# Autodesk Inventor assembly: Ark Test
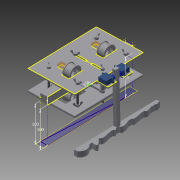
[picture p0: Inventor's stored thumbnail of the model, 180x180]
Saved by Autodesk Inventor 2015 (Build 190159000, 159)
## iProperties
Created: 2018-12-21
Part Number: Ark Test
Document SubType Name: Assembly
Designer: kostya
Author: kostya
## Documents named in this file (12)
- C:\Users\kostya\source\repos\Models\Arkanoid\Ark.ipt\Ark Test.iam
- C:\Users\kostya\source\repos\Models\Arkanoid\Ark.ipt\Top.ipt
- C:\Users\kostya\source\repos\Models\Arkanoid\Ark.ipt\Down.ipt
- C:\Users\kostya\source\repos\Models\Arkanoid\Ark.ipt\Screw.ipt
- C:\Users\kostya\source\repos\Models\Arkanoid\Ark.ipt\Stick.ipt
- C:\Users\kostya\source\repos\Models\Arkanoid\Ark.ipt\Nut.ipt
- C:\Users\kostya\source\repos\Models\Arkanoid\Ark.ipt\Screwk.ipt
- C:\Users\kostya\source\repos\Models\Arkanoid\Ather\ipt\Motors\Servo.ipt
- C:\Users\kostya\source\repos\Models\Arkanoid\Ather\ipt\Motors\Line for servo.ipt
- C:\Users\kostya\source\repos\Models\Arkanoid\Ark.ipt\Wheel.ipt
- C:\Users\kostya\source\repos\Models\Arkanoid\Ark.ipt\Kick.ipt
- C:\Users\kostya\source\repos\Models\Arkanoid\Ark.ipt\Nozzle.ipt
## Components (43 placed, 11 different names)
1. Kick:1 — Вставка:59, Вставка:60, Вставка:61, Вставка:62, Вставка:63, Вставка:64, Вставка:65
2. Nozzle:1 — Вставка:65
3. Top:1 — Вставка:1, Вставка:6, Вставка:7, Вставка:8, Вставка:9, Вставка:15, Вставка:16, Заподлицо:2, Вставка:21, Вставка:22, Вставка:23, Вставка:24, Вставка:46, Вставка:48, Вставка:50, Вставка:51, Вставка:52, Вставка:54, Вставка:55, Заподлицо:7, Совмещение:1, Совмещение:2, Заподлицо:8, Совмещение:3, Совмещение:4
4. Down:1 — Вставка:2, Вставка:3, Вставка:4, Вставка:5, Вставка:10, Вставка:11, Вставка:12, Вставка:13, Заподлицо:1, Заподлицо:2, Вставка:25, Вставка:26, Вставка:27, Вставка:28, Касательность:1, Заподлицо:3, Вставка:47, Вставка:49, Вставка:56, Вставка:57
5. Stick:1 — Заподлицо:1, Касательность:1, Заподлицо:3, Касательность:2, Заподлицо:5, Касательность:3, Касательность:4, Заподлицо:6
6. Nut:1 — Вставка:1, Вставка:36
7. Nut:2 — Вставка:7, Вставка:51
8. Nut:3 — Вставка:6, Вставка:50
9. Nut:4 — Вставка:2
10. Nut:5 — Вставка:4
11. Nut:6 — Вставка:45, Вставка:46
12. Nut:7 — Вставка:5, Вставка:47
13. Nut:8 — Вставка:3, Вставка:49
14. Nut:9 — Вставка:16, Вставка:37
15. Nut:10 — Вставка:15, Вставка:38, Вставка:48
16. Nut:11 — Вставка:8
17. Nut:12 — Вставка:13, Вставка:44
18. Nut:13 — Вставка:10, Вставка:42
19. Nut:14 — Вставка:11, Вставка:40
20. Nut:15 — Вставка:12, Вставка:41
21. Nut:16 — Вставка:9, Вставка:52
22. Nut:17 — Вставка:23
23. Nut:18 — Вставка:24, Вставка:34
24. Nut:19 — Вставка:22
25. Nut:20 — Вставка:21, Вставка:33
26. Nut:21 — Вставка:25
27. Nut:22 — Вставка:26
28. Nut:23 — Вставка:27
29. Nut:24 — Вставка:28
30. Screwk:1 — Вставка:33
31. Screwk:2 — Вставка:34
32. Screw:1 — Вставка:38, Вставка:40
33. Screw:2 — Вставка:37, Вставка:42
34. Screw:3 — Вставка:36, Вставка:41
35. Screw:4 — Вставка:44, Вставка:45
36. Line for servo:2 — Вставка:58, Вставка:59, Вставка:60, Вставка:61
37. Servo:2 — Заподлицо:8, Совмещение:3, Совмещение:4, Вставка:58
38. Servo:1 — Вставка:53, Заподлицо:7, Совмещение:1, Совмещение:2
39. Line for servo:1 — Вставка:53, Вставка:62, Вставка:63, Вставка:64
40. Wheel:1 — Касательность:2, Заподлицо:5, Касательность:3, Вставка:54
41. Wheel:2 — Вставка:57
42. Wheel:3 — Вставка:56
43. Wheel:4 — Вставка:55, Касательность:4, Заподлицо:6
## Relationships (68: Insert 53, Flush 7, Tangent 4, Mate 4)
- Вставка:1 [Insert]: Top:1 ↔ Nut:1
- Вставка:2 [Insert]: Down:1 ↔ Nut:4
- Вставка:3 [Insert]: Down:1 ↔ Nut:8
- Вставка:4 [Insert]: Down:1 ↔ Nut:5
- Вставка:5 [Insert]: Down:1 ↔ Nut:7
- Вставка:6 [Insert]: Top:1 ↔ Nut:3
- Вставка:7 [Insert]: Top:1 ↔ Nut:2
- Вставка:8 [Insert]: Top:1 ↔ Nut:11
- Вставка:9 [Insert]: Top:1 ↔ Nut:16
- Вставка:10 [Insert]: Down:1 ↔ Nut:13
- Вставка:11 [Insert]: Down:1 ↔ Nut:14
- Вставка:12 [Insert]: Down:1 ↔ Nut:15
- Вставка:13 [Insert]: Down:1 ↔ Nut:12
- Вставка:15 [Insert]: Top:1 ↔ Nut:10
- Вставка:16 [Insert]: Top:1 ↔ Nut:9
- Заподлицо:1 [Flush] (32.076 mm): Down:1 ↔ Stick:1
- Заподлицо:2 [Flush]: Top:1 ↔ Down:1
- Вставка:21 [Insert]: Top:1 ↔ Nut:20
- Вставка:22 [Insert]: Top:1 ↔ Nut:19
- Вставка:23 [Insert]: Top:1 ↔ Nut:17
- Вставка:24 [Insert]: Top:1 ↔ Nut:18
- Вставка:25 [Insert]: Down:1 ↔ Nut:21
- Вставка:26 [Insert]: Down:1 ↔ Nut:22
- Вставка:27 [Insert]: Down:1 ↔ Nut:23
- Вставка:28 [Insert]: Down:1 ↔ Nut:24
- Вставка:33 [Insert]: Nut:20 ↔ Screwk:1
- Вставка:34 [Insert]: Nut:18 ↔ Screwk:2
- Касательность:1 [Tangent]: Down:1 ↔ Stick:1
- Заподлицо:3 [Flush]: Down:1 ↔ Stick:1
- Вставка:36 [Insert]: Nut:1 ↔ Screw:3
- Вставка:37 [Insert]: Nut:9 ↔ Screw:2
- Вставка:38 [Insert]: Nut:10 ↔ Screw:1
- Вставка:40 [Insert]: Nut:14 ↔ Screw:1
- Вставка:41 [Insert]: Nut:15 ↔ Screw:3
- Вставка:42 [Insert]: Nut:13 ↔ Screw:2
- Вставка:44 [Insert]: Nut:12 ↔ Screw:4
- Вставка:45 [Insert]: Nut:6 ↔ Screw:4
- Вставка:46 [Insert]: Top:1 ↔ Nut:6
- Вставка:47 [Insert]: Down:1 ↔ Nut:7
- Вставка:48 [Insert]: Top:1 ↔ Nut:10
- Вставка:49 [Insert]: Down:1 ↔ Nut:8
- Вставка:50 [Insert]: Top:1 ↔ Nut:3
- Вставка:51 [Insert]: Top:1 ↔ Nut:2
- Вставка:52 [Insert]: Top:1 ↔ Nut:16
- Вставка:53 [Insert]: Servo:1 ↔ Line for servo:1
- Касательность:2 [Tangent]: Stick:1 ↔ Wheel:1
- Заподлицо:5 [Flush]: Stick:1 ↔ Wheel:1
- Касательность:3 [Tangent]: Stick:1 ↔ Wheel:1
- Вставка:54 [Insert] (-10 mm): Top:1 ↔ Wheel:1
- Вставка:55 [Insert] (-10 mm): Top:1 ↔ Wheel:4
- Касательность:4 [Tangent]: Stick:1 ↔ Wheel:4
- Заподлицо:6 [Flush]: Stick:1 ↔ Wheel:4
- Вставка:56 [Insert] (-23 mm): Down:1 ↔ Wheel:3
- Вставка:57 [Insert] (-23 mm): Down:1 ↔ Wheel:2
- Заподлицо:7 [Flush]: Top:1 ↔ Servo:1
- Совмещение:1 [Mate]: Top:1 ↔ Servo:1
- Совмещение:2 [Mate]: Top:1 ↔ Servo:1
- Заподлицо:8 [Flush]: Top:1 ↔ Servo:2
- Совмещение:3 [Mate]: Top:1 ↔ Servo:2
- Совмещение:4 [Mate]: Top:1 ↔ Servo:2
- Вставка:58 [Insert]: Line for servo:2 ↔ Servo:2
- Вставка:59 [Insert] (2 mm): Kick:1 ↔ Line for servo:2
- Вставка:60 [Insert]: Kick:1 ↔ Line for servo:2
- Вставка:61 [Insert]: Kick:1 ↔ Line for servo:2
- Вставка:62 [Insert]: Kick:1 ↔ Line for servo:1
- Вставка:63 [Insert]: Kick:1 ↔ Line for servo:1
- Вставка:64 [Insert]: Kick:1 ↔ Line for servo:1
- Вставка:65 [Insert]: Kick:1 ↔ Nozzle:1
